# Autodesk Inventor assembly: ENSAMBLAJE_VENTOSA_2
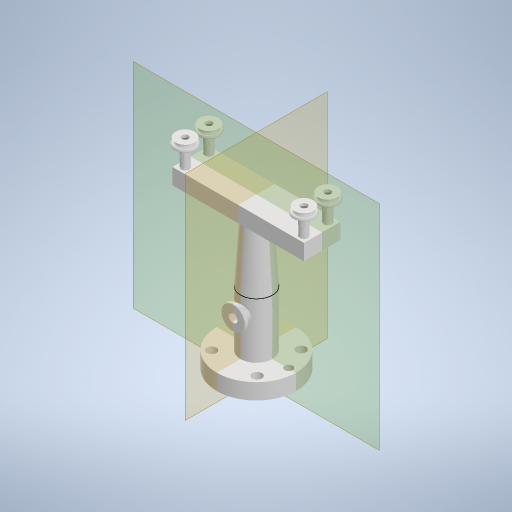
[picture p0: Inventor's stored thumbnail of the model, 512x512]
Saved by Autodesk Inventor 2024 (Build 280153000, 153)
## iProperties
Created: 2022-10-31
Part Number: ENSAMBLAJE_VENTOSA_2
Document SubType Name: Assembly
Designer: Usuario
Mass: 57.9805 g
Surface Area: 254.277 cm^2
Volume: 57.9805 cm^3
Author: Usuario
## Documents named in this file (15)
- C:\Users\sebas\OneDrive\Documentos\Cosas de Sebastian\APM\Esdek\Celda Robotizada\ROBOT STUDIO\CAD\HERRAMIENTA\ENSAMBLAJE_VENTOSA_2.iam
- C:\Users\sebas\OneDrive\Documentos\Cosas de Sebastian\APM\Esdek\Celda Robotizada\ROBOT STUDIO\CAD\HERRAMIENTA\ACOPLE.ipt
- C:\Users\sebas\OneDrive\Documentos\Cosas de Sebastian\APM\Esdek\Celda Robotizada\ROBOT STUDIO\CAD\HERRAMIENTA\TORNILLO_B.ipt
- C:\Users\sebas\OneDrive\Documentos\Cosas de Sebastian\APM\Esdek\Celda Robotizada\ROBOT STUDIO\CAD\HERRAMIENTA\TUBO_METALICO_B.ipt
- C:\Users\sebas\OneDrive\Documentos\Cosas de Sebastian\APM\Esdek\Celda Robotizada\ROBOT STUDIO\CAD\HERRAMIENTA\VENTOSA_B.ipt
- C:\Users\sebas\OneDrive\Documentos\Cosas de Sebastian\APM\Esdek\Celda Robotizada\ROBOT STUDIO\CAD\HERRAMIENTA\UNION_B.ipt
- C:\Users\sebas\OneDrive\Documentos\Cosas de Sebastian\APM\Esdek\Celda Robotizada\ROBOT STUDIO\CAD\HERRAMIENTA\TORNILLO_B_MIR.ipt
- C:\Users\sebas\OneDrive\Documentos\Cosas de Sebastian\APM\Esdek\Celda Robotizada\ROBOT STUDIO\CAD\HERRAMIENTA\TUBO_METALICO_B_MIR.ipt
- C:\Users\sebas\OneDrive\Documentos\Cosas de Sebastian\APM\Esdek\Celda Robotizada\ROBOT STUDIO\CAD\HERRAMIENTA\VENTOSA_B_MIR.ipt
- C:\Users\sebas\OneDrive\Documentos\Cosas de Sebastian\APM\Esdek\Celda Robotizada\ROBOT STUDIO\CAD\HERRAMIENTA\TORNILLO_B_MIR1.ipt
- C:\Users\sebas\OneDrive\Documentos\Cosas de Sebastian\APM\Esdek\Celda Robotizada\ROBOT STUDIO\CAD\HERRAMIENTA\TUBO_METALICO_B_MIR1.ipt
- C:\Users\sebas\OneDrive\Documentos\Cosas de Sebastian\APM\Esdek\Celda Robotizada\ROBOT STUDIO\CAD\HERRAMIENTA\VENTOSA_B_MIR1.ipt
- C:\Users\sebas\OneDrive\Documentos\Cosas de Sebastian\APM\Esdek\Celda Robotizada\ROBOT STUDIO\CAD\HERRAMIENTA\TORNILLO_B_MIR_MIR.ipt
- C:\Users\sebas\OneDrive\Documentos\Cosas de Sebastian\APM\Esdek\Celda Robotizada\ROBOT STUDIO\CAD\HERRAMIENTA\TUBO_METALICO_B_MIR_MIR.ipt
- C:\Users\sebas\OneDrive\Documentos\Cosas de Sebastian\APM\Esdek\Celda Robotizada\ROBOT STUDIO\CAD\HERRAMIENTA\VENTOSA_B_MIR_MIR.ipt
## Components (14 placed, 14 different names)
1. ACOPLE:1 — Nivelación:1, Coincidencia:1, Coincidencia:10
2. TORNILLO_B:4 — Cilíndrica:1, De rotación:2, De rotación:7
3. TUBO_METALICO_B:4 — Cilíndrica:1, Coincidencia:2
4. VENTOSA_B:4 — De rotación:2, Coincidencia:2
5. UNION_B:1 — Nivelación:1, Coincidencia:1, De rotación:7, De rotación:8, De rotación:9, De rotación:10, Coincidencia:9, Coincidencia:11, Coincidencia:12
6. TORNILLO_B_MIR:1 — Cilíndrica:2, De rotación:3, De rotación:9
7. TUBO_METALICO_B_MIR:1 — Coincidencia:3, Cilíndrica:2
8. VENTOSA_B_MIR:1 — Coincidencia:3, De rotación:3
9. TORNILLO_B_MIR1:1 — Cilíndrica:3, De rotación:5, De rotación:8
10. TUBO_METALICO_B_MIR1:1 — Coincidencia:7, Cilíndrica:3
11. VENTOSA_B_MIR1:1 — Coincidencia:7, De rotación:5
12. TORNILLO_B_MIR_MIR:1 — Cilíndrica:4, De rotación:6, De rotación:10
13. TUBO_METALICO_B_MIR_MIR:1 — Coincidencia:8, Cilíndrica:4
14. VENTOSA_B_MIR_MIR:1 — Coincidencia:8, De rotación:6
## Relationships (22: Mate 9, RevoluteJoint 8, CylindricalJoint 4, Flush 1)
- Nivelación:1 [Flush]: ACOPLE:1 ↔ UNION_B:1
- Coincidencia:1 [Mate]: ACOPLE:1 ↔ UNION_B:1
- Cilíndrica:1 [CylindricalJoint]: TORNILLO_B:4 ↔ TUBO_METALICO_B:4
- De rotación:2 [RevoluteJoint] (1 mm): TORNILLO_B:4 ↔ VENTOSA_B:4
- Coincidencia:2 [Mate]: TUBO_METALICO_B:4 ↔ VENTOSA_B:4
- Coincidencia:3 [Mate]: TUBO_METALICO_B_MIR:1 ↔ VENTOSA_B_MIR:1
- Cilíndrica:2 [CylindricalJoint]: TORNILLO_B_MIR:1 ↔ TUBO_METALICO_B_MIR:1
- De rotación:3 [RevoluteJoint] (-1 mm): TORNILLO_B_MIR:1 ↔ VENTOSA_B_MIR:1
- Coincidencia:7 [Mate]: TUBO_METALICO_B_MIR1:1 ↔ VENTOSA_B_MIR1:1
- Coincidencia:8 [Mate]: TUBO_METALICO_B_MIR_MIR:1 ↔ VENTOSA_B_MIR_MIR:1
- Cilíndrica:3 [CylindricalJoint]: TORNILLO_B_MIR1:1 ↔ TUBO_METALICO_B_MIR1:1
- De rotación:5 [RevoluteJoint] (-1 mm): TORNILLO_B_MIR1:1 ↔ VENTOSA_B_MIR1:1
- Cilíndrica:4 [CylindricalJoint]: TORNILLO_B_MIR_MIR:1 ↔ TUBO_METALICO_B_MIR_MIR:1
- De rotación:6 [RevoluteJoint] (1 mm): TORNILLO_B_MIR_MIR:1 ↔ VENTOSA_B_MIR_MIR:1
- De rotación:7 [RevoluteJoint] (4 mm): TORNILLO_B:4 ↔ UNION_B:1
- De rotación:8 [RevoluteJoint] (4 mm): UNION_B:1 ↔ TORNILLO_B_MIR1:1
- De rotación:9 [RevoluteJoint] (4 mm): UNION_B:1 ↔ TORNILLO_B_MIR:1
- De rotación:10 [RevoluteJoint] (4 mm): UNION_B:1 ↔ TORNILLO_B_MIR_MIR:1
- Coincidencia:9 [Mate] (-11.5 mm): UNION_B:1
- Coincidencia:10 [Mate]: ACOPLE:1
- Coincidencia:11 [Mate] (-41.5 mm): UNION_B:1
- Coincidencia:12 [Mate]: UNION_B:1
